# Autodesk Inventor assembly: Sidecar Rev5p2 Assembly
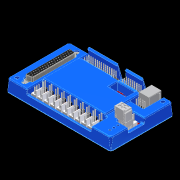
[picture p0: Inventor's stored thumbnail of the model, 180x180]
Saved by Autodesk Inventor 2012 (Build 160160000, 160)
## iProperties
Company: Team 801
Created: 2008-05-31
Part Number: Sidecar Rev5p2 Assembly
Document SubType Name: Assembly
Designer: Jeffrey M
Catalog Web Link: www.team801.org
Author: Jeffrey M
## Documents named in this file (5)
- Z:\UserData\Documents\Inventor\team1885frc\Electronics\DigitalSidecar\elc_Digital_Sidecar_inv.iam
- Z:\UserData\Documents\Inventor\team1885frc\Electronics\DigitalSidecar\Sidecar Rev5 Bottom.ipt
- Z:\UserData\Documents\Inventor\team1885frc\Electronics\DigitalSidecar\Sidecar Rev5 PCB Assembly.iam
- Z:\UserData\Documents\Inventor\team1885frc\Electronics\DigitalSidecar\Wago Power Connector.ipt
- Z:\UserData\Documents\Inventor\team1885frc\Electronics\DigitalSidecar\Sidecar Rev5p2 Top.ipt
## Components (4 placed, 4 different names)
1. Sidecar Rev5 Bottom:1 — Mate:4, Mate:5, Mate:6, Mate:7, Mate:8, Mate:9
2. Sidecar Rev5 PCB Assembly:1 [sub-assembly] — Mate:7, Mate:8, Mate:9, Mate:10, Mate:11, Mate:12
3. Sidecar Rev5p2 Top:1 — Mate:4, Mate:5, Mate:6
4. 734-102:1 — Mate:10, Mate:11, Mate:12
## Relationships (9: Mate 9)
- Mate:4: Sidecar Rev5 Bottom:1 ↔ Sidecar Rev5p2 Top:1
- Mate:5: Sidecar Rev5 Bottom:1 ↔ Sidecar Rev5p2 Top:1
- Mate:6: Sidecar Rev5 Bottom:1 ↔ Sidecar Rev5p2 Top:1
- Mate:7: Sidecar Rev5 Bottom:1 ↔ Sidecar Rev5 PCB Assembly:1
- Mate:8: Sidecar Rev5 Bottom:1 ↔ Sidecar Rev5 PCB Assembly:1
- Mate:9: Sidecar Rev5 Bottom:1 ↔ Sidecar Rev5 PCB Assembly:1
- Mate:10: Sidecar Rev5 PCB Assembly:1 ↔ 734-102:1
- Mate:11: Sidecar Rev5 PCB Assembly:1 ↔ 734-102:1
- Mate:12: Sidecar Rev5 PCB Assembly:1 ↔ 734-102:1
